# Autodesk Inventor assembly: Ball Screw Nut
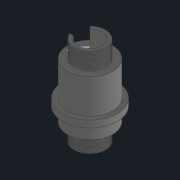
[picture p0: Inventor's stored thumbnail of the model, 180x180]
Saved by Autodesk Inventor 2021 (Build 250183000, 183)
## iProperties
Created: 2020-10-18
Part Number: Ball Screw Nut
Document SubType Name: Assembly
Designer: Eugene Tang
Mass: 217.627 g
Surface Area: 566.46 cm^2
Volume: 217.627 cm^3
Density: 1 g/cm^3
Author: Eugene Tang
## Documents named in this file (4)
- C:\Users\teuge\OneDrive - Curtin University of Technology Australia\Y4S2\DFM\Group Project\CAD\Parts\Assemblies\Ball Screw Nut.iam
- C:\Users\teuge\OneDrive - Curtin University of Technology Australia\Y4S2\DFM\Group Project\CAD\Parts\Ball Screw Nut.ipt
- C:\Users\teuge\OneDrive - Curtin University of Technology Australia\Y4S2\DFM\Group Project\CAD\Parts\Front Return Insert.ipt
- C:\Users\teuge\OneDrive - Curtin University of Technology Australia\Y4S2\DFM\Group Project\CAD\Parts\Rear Return Insert.ipt
## Components (3 placed, 3 different names)
1. Ball Screw Nut:1 — Mate:1, Mate:2, Mate:3, Mate:4, Mate:5, Mate:6
2. Front Return Insert:1 — Mate:1, Mate:5, Mate:6
3. Rear Return Insert:1 — Mate:2, Mate:3, Mate:4
## Relationships (6: Mate 6)
- Mate:1: Ball Screw Nut:1 ↔ Front Return Insert:1
- Mate:2: Ball Screw Nut:1 ↔ Rear Return Insert:1
- Mate:3: Ball Screw Nut:1 ↔ Rear Return Insert:1
- Mate:4: Ball Screw Nut:1 ↔ Rear Return Insert:1
- Mate:5: Ball Screw Nut:1 ↔ Front Return Insert:1
- Mate:6: Ball Screw Nut:1 ↔ Front Return Insert:1
